# Autodesk Inventor assembly: roboticarmassembly
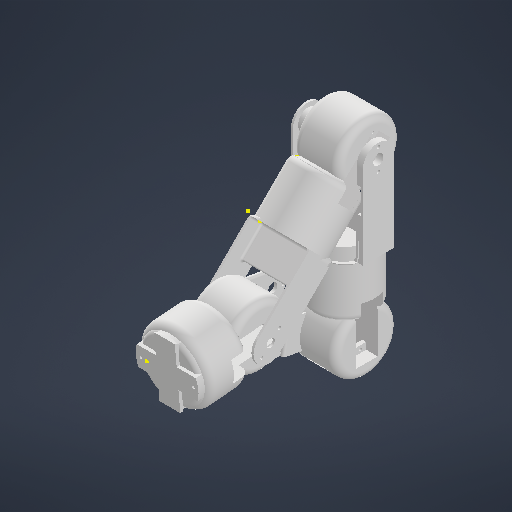
[picture p0: Inventor's stored thumbnail of the model, 512x512]
Saved by Autodesk Inventor 2026.2 (Build 302298000, 298)
## iProperties
Created: 2026-04-09
Part Number: roboticarmassembly
Document SubType Name: Assembly
Designer: Brian Wang
Author: Brian Wang
## Documents named in this file (5)
- C:\Users\Brian Wang\Downloads\RoboticsChess\3D_Model\roboticarmassembly.iam
- C:\Users\Brian Wang\Downloads\RoboticsChess\3D_Model\arm\endpart.ipt
- C:\Users\Brian Wang\Downloads\RoboticsChess\3D_Model\arm\middlepart.ipt
- C:\Users\Brian Wang\Downloads\RoboticsChess\3D_Model\arm\bottomPart.ipt
- C:\Users\Brian Wang\Downloads\RoboticsChess\3D_Model\gripper\main.ipt
## Components (4 placed, 4 different names)
1. endpart:1 — Rotational:2, Rotational:3
2. middlepart:1 — Rotational:1, Rotational:2
3. bottomPart:1 — Rotational:1
4. main:1 — Rotational:3
## Relationships (3: RevoluteJoint 3)
- Rotational:1 [RevoluteJoint]: middlepart:1 ↔ bottomPart:1
- Rotational:2 [RevoluteJoint]: endpart:1 ↔ middlepart:1
- Rotational:3 [RevoluteJoint]: endpart:1 ↔ main:1
